# Autodesk Inventor assembly: main
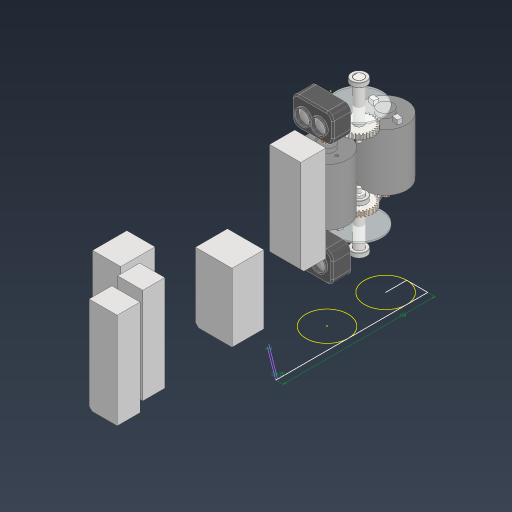
[picture p0: Inventor's stored thumbnail of the model, 512x512]
Saved by Autodesk Inventor 2023 (Build 270158000, 158)
## iProperties
Created: 2026-03-09
Part Number: main
Document SubType Name: Assembly
Designer: szymo
Author: szymo
## Documents named in this file (8)
- D:\tech\robotyka\robots\evangelion-turbo\inventor-project\main.iam
- D:\tech\robotyka\robots\evangelion-turbo\inventor-project\drive-train.iam
- D:\tech\robotyka\robots\evangelion-turbo\inventor-project\LUNA.ipt
- D:\tech\robotyka\robots\evangelion-turbo\inventor-project\2s450mahSHORT.ipt
- D:\tech\robotyka\robots\evangelion-turbo\inventor-project\2s450mah.ipt
- D:\tech\robotyka\robots\evangelion-turbo\inventor-project\3s550mah.ipt
- D:\tech\robotyka\robots\evangelion-turbo\inventor-project\2s550mah.ipt
- D:\tech\robotyka\robots\evangelion-turbo\inventor-project\3s450mah.ipt
## Components (8 placed, 7 different names)
1. drive-train:1 [sub-assembly]
2. LUNA:2
3. LUNA:1
4. 2s450mahSHORT:1
5. 2s450mah:1
6. 3s550mah:1
7. 2s550mah:1
8. 3s450mah:1
## Relationships (1: Flush 1)
- Flush:1 (-101.75 mm)
